# Autodesk Inventor assembly: Doser
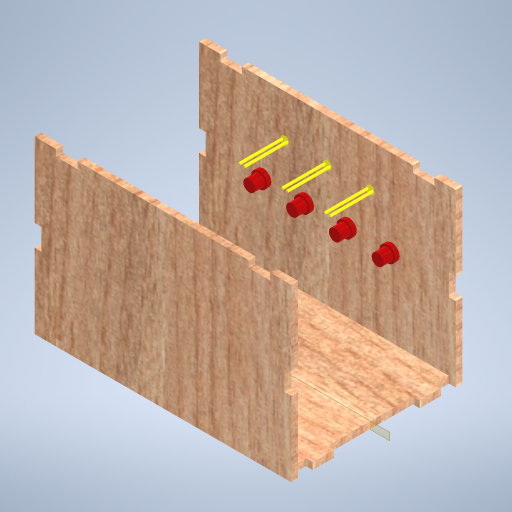
[picture p0: Inventor's stored thumbnail of the model, 512x512]
Saved by Autodesk Inventor 2023.1 (Build 271208000, 208)
## iProperties
Created: 2022-07-13
Part Number: Doser
Document SubType Name: Assembly
Designer: Eli
Author: Eli
## Documents named in this file (6)
- C:\Users\Eli\My Drive\CAD\Resin Doser\Doser.iam
- C:\Users\Eli\My Drive\CAD\Resin Doser\Button.ipt
- C:\Users\Eli\My Drive\CAD\Resin Doser\LED.ipt
- C:\Users\Eli\My Drive\CAD\Resin Doser\Front Panel.ipt
- C:\Users\Eli\My Drive\CAD\Resin Doser\Bottom Panel.ipt
- C:\Users\Eli\My Drive\CAD\Resin Doser\Back Panel.ipt
## Components (10 placed, 5 different names)
1. Front Panel:1 — Mate:1, Flush:1, Mate:2, Mate:3, Flush:2, Flush:3, Angle:1, Angle:2, Angle:3, Mate:4, Mate:5, Mate:6, Mate:7, Mate:8, Mate:9, Mate:10, Mate:11, Mate:12, Mate:13, Flush:4
2. Button:1 — Mate:4, Mate:11
3. LED:1 — Mate:1, Flush:1, Angle:1
4. LED:2 — Mate:3, Flush:2, Angle:3
5. LED:3 — Mate:2, Flush:3, Angle:2
6. Button:2 — Mate:7, Mate:8
7. Button:3 — Mate:6, Mate:9
8. Button:4 — Mate:5, Mate:10
9. Bottom Panel:1 — Mate:12, Mate:13, Flush:4
10. Back Panel:1
## Relationships (20: Mate 13, Flush 4, Angle 3)
- Mate:1: Front Panel:1 ↔ LED:1
- Flush:1: Front Panel:1 ↔ LED:1
- Mate:2: Front Panel:1 ↔ LED:3
- Mate:3: Front Panel:1 ↔ LED:2
- Flush:2: Front Panel:1 ↔ LED:2
- Flush:3: Front Panel:1 ↔ LED:3
- Angle:1 (0 deg): Front Panel:1 ↔ LED:1
- Angle:2 (0 deg): Front Panel:1 ↔ LED:3
- Angle:3 (0 deg): Front Panel:1 ↔ LED:2
- Mate:4: Front Panel:1 ↔ Button:1
- Mate:5: Front Panel:1 ↔ Button:4
- Mate:6: Front Panel:1 ↔ Button:3
- Mate:7: Front Panel:1 ↔ Button:2
- Mate:8: Front Panel:1 ↔ Button:2
- Mate:9: Front Panel:1 ↔ Button:3
- Mate:10: Front Panel:1 ↔ Button:4
- Mate:11: Front Panel:1 ↔ Button:1
- Mate:12: Front Panel:1 ↔ Bottom Panel:1
- Mate:13: Front Panel:1 ↔ Bottom Panel:1
- Flush:4: Front Panel:1 ↔ Bottom Panel:1
